# Autodesk Inventor assembly: CCM_Unit
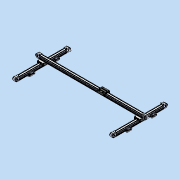
[picture p0: Inventor's stored thumbnail of the model, 180x180]
Saved by Autodesk Inventor 2020 (Build 240168000, 168)
## iProperties
Created: 2021-02-24
Part Number: CCM_Unit
Document SubType Name: Assembly
Designer: magnarecta
Author: magnarecta
## Documents named in this file (5)
- C:\Users\lvglv\Documents\GitHub\Eto_Project\Hardware\Asem\CCM_Unit.iam
- C:\Users\lvglv\Documents\GitHub\Eto_Project\Hardware\Parts\CCM\CCM motion linear guide rail\CCM_UNIT\CCM_Unit_C.iam
- C:\Users\lvglv\Documents\GitHub\Eto_Project\Hardware\Parts\CCM\CCM motion linear guide rail\CCM_UNIT\CCM_Unit_A.iam
- C:\Users\lvglv\Documents\GitHub\Eto_Project\Hardware\Parts\CCM\CCM motion linear guide rail\CCM_UNIT\CCM_Unit_B.iam
- C:\Users\lvglv\Documents\GitHub\Eto_Project\Hardware\Parts\Meviy\CCM_Mount_A.ipt
## Components (5 placed, 4 different names)
1. CCM_Unit_C:1 [sub-assembly] — メイト:1, 角度:1, メイト:2, フラッシュ:5, フラッシュ:6, メイト:3, フラッシュ:8
2. CCM_Unit_A:1 [sub-assembly] — フラッシュ:1, フラッシュ:2, フラッシュ:3, フラッシュ:4, メイト:1, 角度:1, 挿入:3, 挿入:4
3. CCM_Unit_B:1 [sub-assembly] — フラッシュ:1, フラッシュ:2, フラッシュ:3, フラッシュ:4, 挿入:1, 挿入:2
4. CCM_Mount_A:1 — メイト:2, フラッシュ:5, 挿入:1, 挿入:2, フラッシュ:6, フラッシュ:7
5. CCM_Mount_A:2 — メイト:3, フラッシュ:7, 挿入:3, 挿入:4, フラッシュ:8
## Relationships (16: Flush 8, Insert 4, Mate 3, Angle 1)
- フラッシュ:1 [Flush]: CCM_Unit_A:1 ↔ CCM_Unit_B:1
- フラッシュ:2 [Flush]: CCM_Unit_A:1 ↔ CCM_Unit_B:1
- フラッシュ:3 [Flush]: CCM_Unit_A:1 ↔ CCM_Unit_B:1
- フラッシュ:4 [Flush]: CCM_Unit_A:1 ↔ CCM_Unit_B:1
- メイト:1 [Mate] (3 mm): CCM_Unit_C:1 ↔ CCM_Unit_A:1
- 角度:1 [Angle] (0 deg): CCM_Unit_C:1 ↔ CCM_Unit_A:1
- メイト:2 [Mate]: CCM_Unit_C:1 ↔ CCM_Mount_A:1
- フラッシュ:5 [Flush] (-20 mm): CCM_Unit_C:1 ↔ CCM_Mount_A:1
- 挿入:1 [Insert]: CCM_Unit_B:1 ↔ CCM_Mount_A:1
- 挿入:2 [Insert]: CCM_Unit_B:1 ↔ CCM_Mount_A:1
- フラッシュ:6 [Flush]: CCM_Unit_C:1 ↔ CCM_Mount_A:1
- メイト:3 [Mate]: CCM_Unit_C:1 ↔ CCM_Mount_A:2
- フラッシュ:7 [Flush]: CCM_Mount_A:1 ↔ CCM_Mount_A:2
- 挿入:3 [Insert]: CCM_Unit_A:1 ↔ CCM_Mount_A:2
- 挿入:4 [Insert]: CCM_Unit_A:1 ↔ CCM_Mount_A:2
- フラッシュ:8 [Flush]: CCM_Unit_C:1 ↔ CCM_Mount_A:2
